# Autodesk Inventor assembly: SmoothieBox
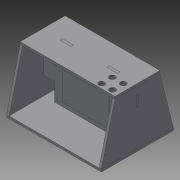
[picture p0: Inventor's stored thumbnail of the model, 180x180]
Saved by Autodesk Inventor 2014 (Build 180170000, 170)
## iProperties
Created: 2015-02-09
Part Number: SmoothieBox
Document SubType Name: Assembly
Designer: ThatOtherGuy
Author: ThatOtherGuy
## Documents named in this file (7)
- C:\Users\ThatOtherGuy\Documents\Inventor\KosselCNC1515\ElectronicsSmoothie\SmoothieBox.iam
- C:\Users\ThatOtherGuy\Documents\Inventor\KosselCNC1515\ElectronicsSmoothie\Center_Mount.ipt
- C:\Users\ThatOtherGuy\Documents\Inventor\KosselCNC1515\ElectronicsSmoothie\Base.ipt
- C:\Users\ThatOtherGuy\Documents\Inventor\KosselCNC1515\ElectronicsSmoothie\Side.ipt
- C:\Users\ThatOtherGuy\Documents\Inventor\KosselCNC1515\12V20A_PowerSupply.ipt
- C:\Users\ThatOtherGuy\Documents\Inventor\KosselCNC1515\ElectronicsSmoothie\Top.ipt
- C:\Users\ThatOtherGuy\Documents\Inventor\KosselCNC1515\ElectronicsSmoothie\Smoothieboard.ipt
## Components (7 placed, 6 different names)
1. Center_Mount:1 — Mate:1, Mate:2, Mate:3, Mate:4, Mate:5, Mate:6, Mate:7, Mate:8, Mate:9, Mate:12, Mate:13, Mate:14, Mate:15, Insert:1, Insert:2
2. Base:1 — Mate:1, Mate:2, Mate:3, Mate:10
3. Side:1 — Mate:7, Mate:8, Mate:9, Mate:11
4. Side:2 — Mate:4, Mate:5, Mate:6
5. 12V20A_PowerSupply:1 — Mate:10, Mate:11, Mate:12
6. Top:1 — Mate:13, Mate:14, Mate:15
7. Smoothieboard:1 — Insert:1, Insert:2
## Relationships (17: Mate 15, Insert 2)
- Mate:1: Center_Mount:1 ↔ Base:1
- Mate:2: Center_Mount:1 ↔ Base:1
- Mate:3: Center_Mount:1 ↔ Base:1
- Mate:4: Center_Mount:1 ↔ Side:2
- Mate:5: Center_Mount:1 ↔ Side:2
- Mate:6: Center_Mount:1 ↔ Side:2
- Mate:7: Center_Mount:1 ↔ Side:1
- Mate:8: Center_Mount:1 ↔ Side:1
- Mate:9: Center_Mount:1 ↔ Side:1
- Mate:10: Base:1 ↔ 12V20A_PowerSupply:1
- Mate:11: Side:1 ↔ 12V20A_PowerSupply:1
- Mate:12: Center_Mount:1 ↔ 12V20A_PowerSupply:1
- Mate:13: Center_Mount:1 ↔ Top:1
- Mate:14: Center_Mount:1 ↔ Top:1
- Mate:15: Center_Mount:1 ↔ Top:1
- Insert:1 (10 mm): Center_Mount:1 ↔ Smoothieboard:1
- Insert:2 (10 mm): Center_Mount:1 ↔ Smoothieboard:1
